# Autodesk Inventor assembly: Assembly1
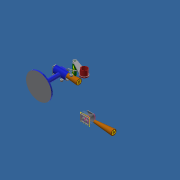
[picture p0: Inventor's stored thumbnail of the model, 180x180]
Saved by Autodesk Inventor 2018 (Build 220112000, 112)
## iProperties
Created: 2022-02-21
Part Number: Assembly1
Document SubType Name: Assembly
Designer: Nathann
Author: Nathann
## Documents named in this file (14)
- C:\Users\Nathann\OneDrive\Objet3D\EPFLEplucheCarrote\Assembly1.iam
- C:\Users\Nathann\OneDrive\Objet3D\EPFLEplucheCarrote\Feet.ipt
- C:\Users\Nathann\OneDrive\Objet3D\EPFLEplucheCarrote\Manivelle.ipt
- C:\Users\Nathann\OneDrive\Objet3D\EPFLEplucheCarrote\Handle.ipt
- C:\Users\Nathann\OneDrive\Objet3D\EPFLEplucheCarrote\Carrote.ipt
- C:\Users\Nathann\OneDrive\Objet3D\EPFLEplucheCarrote\Carrot_Peeler_Blade.ipt
- C:\Users\Nathann\OneDrive\Objet3D\FaucetLaminarFlow\CarrotRoller.ipt
- C:\Users\Nathann\OneDrive\Objet3D\FaucetLaminarFlow\SpringLoadedRollerHolder.ipt
- C:\Users\Nathann\OneDrive\Objet3D\FaucetLaminarFlow\BladeHolderSpringLoaded.ipt
- C:\Users\Nathann\OneDrive\Objet3D\FaucetLaminarFlow\CarrotPeelerBodyV2.ipt
- C:\Users\Nathann\OneDrive\Objet3D\FaucetLaminarFlow\CarrotPeelerBodyCoverV2.ipt
- C:\Users\Nathann\OneDrive\Objet3D\FaucetLaminarFlow\RollerMecanumHolder.ipt
- C:\Users\Nathann\OneDrive\Objet3D\FaucetLaminarFlow\CarrotMecanumRoller.ipt
- C:\Users\Nathann\OneDrive\Objet3D\FaucetLaminarFlow\MecanumRollerPin.ipt
## Components (19 placed, 13 different names)
1. Feet:1 — Mate:2, Mate:5, Mate:6, Flush:5
2. Manivelle:1 — Flush:2
3. Handle:1 — Flush:2
4. Carrote:1 — Mate:2
5. Carrot_Peeler_Blade:1 — Mate:3, Insert:2, Flush:3
6. CarrotRoller:1
7. SpringLoadedRollerHolder:1 — Mate:5
8. BladeHolderSpringLoaded:1 — Mate:3, Insert:2, Flush:3, Mate:4, Angle:1, Flush:4, Mate:6
9. Carrot_Peeler_Blade:2 — Insert:3, Insert:4
10. CarrotRoller:2
11. Carrot_Peeler_Blade:16
12. CarrotPeelerBodyV2:1 — Insert:3, Insert:4
13. CarrotPeelerBodyCoverV2:1
14. RollerMecanumHolder:1 — Insert:5, Insert:6
15. CarrotMecanumRoller:1 — Mate:8
16. CarrotMecanumRoller:2 — Mate:7
17. MecanumRollerPin:1 — Insert:6, Mate:7
18. MecanumRollerPin:2 — Insert:5, Mate:8
19. Carrote:2
## Relationships (17: Mate 7, Insert 5, Flush 4, Angle 1)
- Flush:2: Manivelle:1 ↔ Handle:1
- Mate:2: Feet:1 ↔ Carrote:1
- Mate:3: Carrot_Peeler_Blade:1 ↔ BladeHolderSpringLoaded:1
- Insert:2: Carrot_Peeler_Blade:1 ↔ BladeHolderSpringLoaded:1
- Flush:3: Carrot_Peeler_Blade:1 ↔ BladeHolderSpringLoaded:1
- Mate:4: BladeHolderSpringLoaded:1
- Angle:1 (45 deg): BladeHolderSpringLoaded:1
- Flush:4: BladeHolderSpringLoaded:1
- Mate:5: Feet:1 ↔ SpringLoadedRollerHolder:1
- Mate:6: Feet:1 ↔ BladeHolderSpringLoaded:1
- Flush:5: Feet:1
- Insert:3: Carrot_Peeler_Blade:2 ↔ CarrotPeelerBodyV2:1
- Insert:4: Carrot_Peeler_Blade:2 ↔ CarrotPeelerBodyV2:1
- Insert:5: RollerMecanumHolder:1 ↔ MecanumRollerPin:2
- Insert:6: RollerMecanumHolder:1 ↔ MecanumRollerPin:1
- Mate:7: CarrotMecanumRoller:2 ↔ MecanumRollerPin:1
- Mate:8: CarrotMecanumRoller:1 ↔ MecanumRollerPin:2
